# Autodesk Inventor assembly: ワイヤジンバル
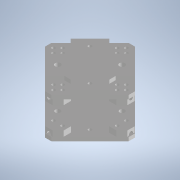
[picture p0: Inventor's stored thumbnail of the model, 180x180]
Saved by Autodesk Inventor 2020 (Build 240168000, 168)
## iProperties
Created: 2019-10-22
Part Number: ワイヤジンバル
Document SubType Name: Assembly
Designer: highs
Author: highs
## Documents named in this file (4)
- C:\Users\highs\Desktop\タスク\現在のタスク\中の島ex\ワイヤジンバル.iam
- C:\Users\highs\Desktop\タスク\現在のタスク\中の島ex\ワイヤジンバル1.ipt
- C:\Users\highs\Desktop\タスク\現在のタスク\中の島ex\ワイヤジンバル2.ipt
- C:\Users\highs\Desktop\タスク\現在のタスク\中の島ex\ワイヤジンバル3.ipt
## Components (10 placed, 3 different names)
1. ワイヤジンバル1:1 — メイト:1, メイト:2, メイト:3, メイト:4, メイト:5, メイト:9, メイト:10, メイト:11, メイト:12, メイト:13, メイト:14, メイト:15, メイト:16, メイト:17
2. ワイヤジンバル2:1 — メイト:4, メイト:5, メイト:6, メイト:7, メイト:8, メイト:18, メイト:19, メイト:20, メイト:21, メイト:22, メイト:23, メイト:24, メイト:25, メイト:26
3. ワイヤジンバル3:1 — メイト:1, メイト:2, メイト:3
4. ワイヤジンバル3:2 — メイト:6, メイト:7, メイト:8
5. ワイヤジンバル3:3 — メイト:9, メイト:10, メイト:11
6. ワイヤジンバル3:4 — メイト:15, メイト:16, メイト:17
7. ワイヤジンバル3:5 — メイト:12, メイト:13, メイト:14
8. ワイヤジンバル3:6 — メイト:18, メイト:19, メイト:20
9. ワイヤジンバル3:7 — メイト:21, メイト:22, メイト:23
10. ワイヤジンバル3:8 — メイト:24, メイト:25, メイト:26
## Relationships (26: Mate 26)
- メイト:1 [Mate]: ワイヤジンバル1:1 ↔ ワイヤジンバル3:1
- メイト:2 [Mate]: ワイヤジンバル1:1 ↔ ワイヤジンバル3:1
- メイト:3 [Mate]: ワイヤジンバル1:1 ↔ ワイヤジンバル3:1
- メイト:4 [Mate]: ワイヤジンバル1:1 ↔ ワイヤジンバル2:1
- メイト:5 [Mate]: ワイヤジンバル1:1 ↔ ワイヤジンバル2:1
- メイト:6 [Mate]: ワイヤジンバル2:1 ↔ ワイヤジンバル3:2
- メイト:7 [Mate]: ワイヤジンバル2:1 ↔ ワイヤジンバル3:2
- メイト:8 [Mate]: ワイヤジンバル2:1 ↔ ワイヤジンバル3:2
- メイト:9 [Mate]: ワイヤジンバル1:1 ↔ ワイヤジンバル3:3
- メイト:10 [Mate]: ワイヤジンバル1:1 ↔ ワイヤジンバル3:3
- メイト:11 [Mate]: ワイヤジンバル1:1 ↔ ワイヤジンバル3:3
- メイト:12 [Mate]: ワイヤジンバル1:1 ↔ ワイヤジンバル3:5
- メイト:13 [Mate]: ワイヤジンバル1:1 ↔ ワイヤジンバル3:5
- メイト:14 [Mate]: ワイヤジンバル1:1 ↔ ワイヤジンバル3:5
- メイト:15 [Mate]: ワイヤジンバル1:1 ↔ ワイヤジンバル3:4
- メイト:16 [Mate]: ワイヤジンバル1:1 ↔ ワイヤジンバル3:4
- メイト:17 [Mate]: ワイヤジンバル1:1 ↔ ワイヤジンバル3:4
- メイト:18 [Mate]: ワイヤジンバル2:1 ↔ ワイヤジンバル3:6
- メイト:19 [Mate]: ワイヤジンバル2:1 ↔ ワイヤジンバル3:6
- メイト:20 [Mate]: ワイヤジンバル2:1 ↔ ワイヤジンバル3:6
- メイト:21 [Mate]: ワイヤジンバル2:1 ↔ ワイヤジンバル3:7
- メイト:22 [Mate]: ワイヤジンバル2:1 ↔ ワイヤジンバル3:7
- メイト:23 [Mate]: ワイヤジンバル2:1 ↔ ワイヤジンバル3:7
- メイト:24 [Mate]: ワイヤジンバル2:1 ↔ ワイヤジンバル3:8
- メイト:25 [Mate]: ワイヤジンバル2:1 ↔ ワイヤジンバル3:8
- メイト:26 [Mate]: ワイヤジンバル2:1 ↔ ワイヤジンバル3:8
